# Autodesk Inventor assembly: EnsambleFinalSim
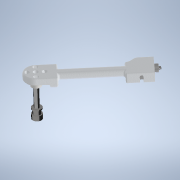
[picture p0: Inventor's stored thumbnail of the model, 180x180]
Saved by Autodesk Inventor 2021 (Build 250183000, 183)
## iProperties
Created: 2022-10-27
Part Number: EnsambleFinalSim
Document SubType Name: Assembly
Designer: zulet
Author: zulet
## Documents named in this file (19)
- D:\UNAL\2022-2S\Servomecanismos\Proyecto Academico\Servomecanismo2R-main\Servomecanismo2R\INVENTOR\Piezas3D\Piezas3D\EnsambleFinalSim.iam
- D:\UNAL\2022-2S\Servomecanismos\Proyecto Academico\Motorreductor.ipt
- D:\UNAL\2022-2S\Servomecanismos\Proyecto Academico\Acople4a8.ipt
- D:\UNAL\2022-2S\Servomecanismos\Proyecto Academico\Polea.ipt
- D:\UNAL\2022-2S\Servomecanismos\Proyecto Academico\Eje8.ipt
- C:\Users\zulet\OneDrive\Documents\Inventor\Content Center Files\R2021\en-US\BS 290 SKF(20)\BS 290 SKF - SKF 608-2RZ.ipt
- D:\UNAL\2022-2S\Servomecanismos\Proyecto Academico\Servomecanismo2R-main\Servomecanismo2R\INVENTOR\Piezas3D\Piezas3D\Eslabon1.ipt
- D:\UNAL\2022-2S\Servomecanismos\Proyecto Academico\Servomecanismo2R-main\Servomecanismo2R\INVENTOR\Piezas3D\Piezas3D\Eslabon2.ipt
- D:\UNAL\2022-2S\Servomecanismos\Proyecto Academico\Servomecanismo2R-main\Servomecanismo2R\INVENTOR\Piezas3D\Piezas3D\Eje.ipt
- D:\UNAL\2022-2S\Servomecanismos\Proyecto Academico\Servomecanismo2R-main\Servomecanismo2R\INVENTOR\Piezas3D\Piezas3D\Tensor.ipt
- D:\UNAL\2022-2S\Servomecanismos\Proyecto Academico\AcopleBrida4.ipt
- D:\UNAL\2022-2S\Servomecanismos\Proyecto Academico\AcopleBrida8mm.ipt
- D:\UNAL\2022-2S\Servomecanismos\Proyecto Academico\Servomecanismo2R-main\Servomecanismo2R\INVENTOR\Piezas3D\Piezas3D\Tower Pro MG90S Micro servo\Tower Pro MG90S Micro servo.iam
- D:\UNAL\2022-2S\Servomecanismos\Proyecto Academico\Servomecanismo2R-main\Servomecanismo2R\INVENTOR\Piezas3D\Piezas3D\BaseM1.ipt
- D:\UNAL\2022-2S\Servomecanismos\Proyecto Academico\Servomecanismo2R-main\Servomecanismo2R\INVENTOR\Piezas3D\Piezas3D\SoporteMarcador.ipt
- D:\UNAL\2022-2S\Servomecanismos\Proyecto Academico\Servomecanismo2R-main\Servomecanismo2R\INVENTOR\Piezas3D\Piezas3D\PortaMarcador.ipt
- D:\UNAL\2022-2S\Servomecanismos\Proyecto Academico\Servomecanismo2R-main\Servomecanismo2R\INVENTOR\Piezas3D\Piezas3D\PlacaBase.ipt
- D:\UNAL\2022-2S\Servomecanismos\Proyecto Academico\Servomecanismo2R-main\Servomecanismo2R\INVENTOR\Piezas3D\Piezas3D\marcador.ipt
- C:\Users\zulet\OneDrive\Documents\Inventor\Content Center Files\R2021\en-US\DIN 7985 (H)\DIN 7985 (H) - M2x6-H.ipt
## Components (22 placed, 18 different names)
1. Motorreductor:1 — Rigid:1, Rigid:7
2. Acople4a8:1 — Rigid:5, Rigid:7
3. Eje8:1 — Rigid:5, Rigid:6
4. BS 290 SKF- with two low-friction seals SKF 608-2RZ:1 — Rigid:9
5. Eslabon1:1 — Rigid:8, Rigid:9, Rigid:10
6. Polea:3 — Rigid:6
7. AcopleBrida4:1 — Rigid:8
8. Motorreductor:2 — Rigid:2
9. SoporteMarcador:1
10. PlacaBase:1 — Rigid:3, Rigid:4
11. BaseM1:1 — Rigid:1, Rigid:4
12. BaseM1:2 — Rigid:2, Rigid:3
13. Eslabon2:1
14. Tensor:1 — Rigid:10, Rigid:11
15. Eje:1
16. Polea:4
17. BS 290 SKF- with two low-friction seals SKF 608-2RZ:2 — Rigid:11
18. AcopleBrida8mm:1
19. Tower Pro MG90S Micro servo:1 [sub-assembly]
20. PortaMarcador:1
21. marcador:1
22. DIN 7985 (H) M2x6-H:1
## Relationships (11: WeldJoint 11)
- Rigid:1 [WeldJoint]: Motorreductor:1 ↔ BaseM1:1
- Rigid:2 [WeldJoint]: Motorreductor:2 ↔ BaseM1:2
- Rigid:3 [WeldJoint]: PlacaBase:1 ↔ BaseM1:2
- Rigid:4 [WeldJoint]: PlacaBase:1 ↔ BaseM1:1
- Rigid:5 [WeldJoint]: Acople4a8:1 ↔ Eje8:1
- Rigid:6 [WeldJoint] (5 mm): Eje8:1 ↔ Polea:3
- Rigid:7 [WeldJoint]: Motorreductor:1 ↔ Acople4a8:1
- Rigid:8 [WeldJoint]: Eslabon1:1 ↔ AcopleBrida4:1
- Rigid:9 [WeldJoint]: BS 290 SKF- with two low-friction seals SKF 608-2RZ:1 ↔ Eslabon1:1
- Rigid:10 [WeldJoint] (-7.5 mm): Eslabon1:1 ↔ Tensor:1
- Rigid:11 [WeldJoint]: Tensor:1 ↔ BS 290 SKF- with two low-friction seals SKF 608-2RZ:2
